# Autodesk Inventor assembly: Крышка
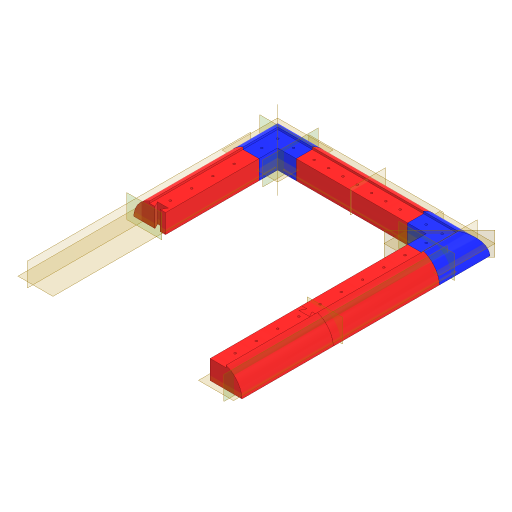
[picture p0: Inventor's stored thumbnail of the model, 512x512]
Saved by Autodesk Inventor 2023.2 (Build 272271030, 271C)
## iProperties
Created: 2025-05-05
Part Number: Крышка
Document SubType Name: Assembly
Designer: Олег Коноваленко
Author: Олег Коноваленко
## Documents named in this file (4)
- D:\!Rover\Rover\Rover_construction\Крышка.iam
- D:\!Rover\Rover\Rover_construction\Край задней части корпуса.ipt
- D:\!Rover\Rover\Rover_construction\кубик.ipt
- D:\!Rover\Rover\Rover_construction\Фанера_крышки.ipt
## Components (6 placed, 3 different names)
1. Край задней части корпуса:1 — Совмещение:1, Заподлицо:1, Совмещение:2, Совмещение:5, Заподлицо:3, Заподлицо:4
2. Край задней части корпуса:2 — Совмещение:6, Заподлицо:5, Заподлицо:6, Совмещение:8
3. Край задней части корпуса:3 — Совмещение:3, Заподлицо:2, Совмещение:4, Совмещение:7
4. кубик:1 — Совмещение:1, Заподлицо:1, Совмещение:2, Совмещение:3, Заподлицо:2, Совмещение:4
5. кубик:2 — Совмещение:5, Заподлицо:3, Заподлицо:4, Совмещение:6, Заподлицо:5, Заподлицо:6, Совмещение:9
6. Фанера_крышки:1 — Совмещение:7, Совмещение:8, Совмещение:9
## Relationships (15: Mate 9, Flush 6)
- Совмещение:1 [Mate]: Край задней части корпуса:1 ↔ кубик:1
- Заподлицо:1 [Flush]: Край задней части корпуса:1 ↔ кубик:1
- Совмещение:2 [Mate]: Край задней части корпуса:1 ↔ кубик:1
- Совмещение:3 [Mate]: Край задней части корпуса:3 ↔ кубик:1
- Заподлицо:2 [Flush]: Край задней части корпуса:3 ↔ кубик:1
- Совмещение:4 [Mate]: Край задней части корпуса:3 ↔ кубик:1
- Совмещение:5 [Mate]: Край задней части корпуса:1 ↔ кубик:2
- Заподлицо:3 [Flush]: Край задней части корпуса:1 ↔ кубик:2
- Заподлицо:4 [Flush]: Край задней части корпуса:1 ↔ кубик:2
- Совмещение:6 [Mate]: Край задней части корпуса:2 ↔ кубик:2
- Заподлицо:5 [Flush]: Край задней части корпуса:2 ↔ кубик:2
- Заподлицо:6 [Flush]: Край задней части корпуса:2 ↔ кубик:2
- Совмещение:7 [Mate]: Край задней части корпуса:3 ↔ Фанера_крышки:1
- Совмещение:8 [Mate]: Край задней части корпуса:2 ↔ Фанера_крышки:1
- Совмещение:9 [Mate]: кубик:2 ↔ Фанера_крышки:1
